# Autodesk Inventor assembly: plugassmbly
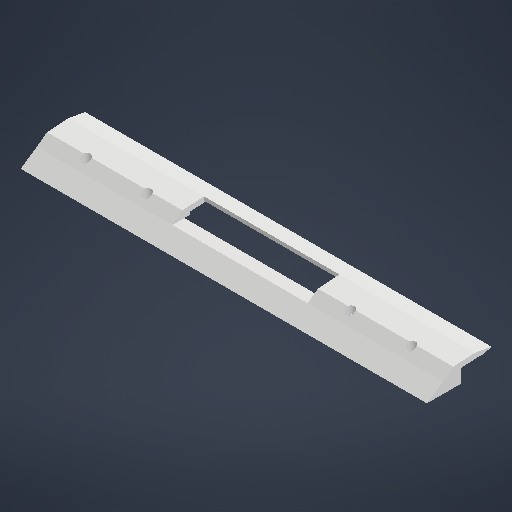
[picture p0: Inventor's stored thumbnail of the model, 512x512]
Saved by Autodesk Inventor 2026.2 (Build 302298010, 298A)
## iProperties
Created: 2026-05-09
Part Number: plugassmbly
Document SubType Name: Assembly
Designer: karol
Author: karol
## Documents named in this file (4)
- C:\Users\karol\OneDrive\Dokumenty\GitHub\bolt\bolt\cad\assembly\plugassmbly.iam
- C:\Users\karol\OneDrive\Dokumenty\GitHub\bolt\bolt\cad\ready parts\pługmoj.ipt
- C:\Users\karol\OneDrive\Dokumenty\GitHub\bolt\bolt\cad\ready parts\mocowanie do pługu.ipt
- C:\Users\karol\OneDrive\Dokumenty\GitHub\bolt\bolt\cad\ready parts\przódv3.ipt
## Components (3 placed, 3 different names)
1. pługmoj:1 — Mate:1, Mate:2, Mate:3, Flush:1
2. mocowanie do pługu:1 — Mate:1, Mate:2, Mate:3, Mate:4, Flush:2
3. przódv3:1 — Mate:4, Flush:1, Flush:2
## Relationships (6: Mate 4, Flush 2)
- Mate:1: pługmoj:1 ↔ mocowanie do pługu:1
- Mate:2: pługmoj:1 ↔ mocowanie do pługu:1
- Mate:3: pługmoj:1 ↔ mocowanie do pługu:1
- Mate:4: mocowanie do pługu:1 ↔ przódv3:1
- Flush:1: pługmoj:1 ↔ przódv3:1
- Flush:2: mocowanie do pługu:1 ↔ przódv3:1
